# Autodesk Inventor assembly: Сборка
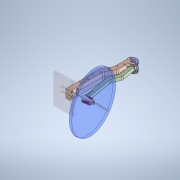
[picture p0: Inventor's stored thumbnail of the model, 180x180]
Saved by Autodesk Inventor 2021.2 (Build 252289000, 289)
## iProperties
Created: 2024-10-29
Part Number: Сборка
Document SubType Name: Assembly
Designer: barko
Author: barko
## Documents named in this file (14)
- C:\Users\barko\Desktop\Daniil\MIET\PID_controller\Mechanics\3D_model\Сборка.iam
- C:\Users\barko\Desktop\Daniil\MIET\PID_controller\Mechanics\3D_model\Ножка 1.ipt
- C:\Users\barko\Desktop\Daniil\MIET\PID_controller\Mechanics\3D_model\Ножка 2.ipt
- C:\Users\barko\Desktop\Daniil\MIET\PID_controller\Mechanics\3D_model\Скобка 1.ipt
- C:\Users\barko\Desktop\Daniil\MIET\PID_controller\Mechanics\3D_model\Скобка 2.ipt
- C:\Users\barko\Desktop\Daniil\MIET\PID_controller\Mechanics\3D_model\Фланец.ipt
- C:\Users\barko\Desktop\Daniil\MIET\PID_controller\Mechanics\3D_model\Луч.ipt
- C:\Users\barko\Desktop\Daniil\MIET\PID_controller\Mechanics\3D_model\Ложечка.ipt
- C:\Users\barko\Desktop\Daniil\MIET\PID_controller\Mechanics\3D_model\Моторчик.ipt
- C:\Users\barko\Desktop\Daniil\MIET\PID_controller\Mechanics\3D_model\Пропеллер.ipt
- C:\Users\barko\Documents\Inventor\Content Center Files\R2021\ru-RU\GOST 11738-84\Винт M3-6gx30 ГОСТ 11738-84.ipt
- C:\Users\barko\Documents\Inventor\Content Center Files\R2021\ru-RU\GOST 5916-70\Гайка M3-6H ГОСТ 5916-70.ipt
- C:\Users\barko\Documents\Inventor\Content Center Files\R2021\ru-RU\Nut GOST 15524-70\Гайка M4-6H ГОСТ 15524-70.ipt
- C:\Users\barko\Documents\Inventor\Content Center Files\R2021\ru-RU\GOST 11738-84\Винт M4-6gx25 ГОСТ 11738-84.ipt
## Components (25 placed, 13 different names)
1. Ножка 1:1 — Совмещение:1, Угол:1, Совмещение:2, Совмещение:3, Совмещение:4, Совмещение:5, Совмещение:6, Совмещение:7, Совмещение:8, Совмещение:9, Совмещение:10, Совмещение:11, Совмещение:12, Совмещение:13, Совмещение:14, Совмещение:15, Совмещение:16, Совмещение:18, Совмещение:20, Совмещение:22, Совмещение:24, Совмещение:26, Совмещение:28, Совмещение:33, Касательность:1, Касательность:2
2. Ножка 2:1 — Совмещение:17, Совмещение:19, Совмещение:21, Совмещение:23, Совмещение:25, Совмещение:27, Совмещение:29
3. Скобка 1:1 — Совмещение:34
4. Скобка 2:1
5. Фланец:1
6. Луч:1 — Вставка:3, Заподлицо:1, Совмещение:1, Угол:1
7. Ложечка:1 — Вставка:1
8. Моторчик:1 — Вставка:1, Вставка:2, Вставка:3
9. Пропеллер:1 — Вставка:2
10. Винт ГОСТ 11738-84 M 3x30:1 — Совмещение:2, Совмещение:3
11. Гайка ГОСТ 5916-70 M3:1 — Совмещение:16, Совмещение:17
12. Винт ГОСТ 11738-84 M 3x30:2 — Совмещение:4, Совмещение:5
13. Винт ГОСТ 11738-84 M 3x30:3 — Совмещение:6, Совмещение:7
14. Винт ГОСТ 11738-84 M 3x30:4 — Совмещение:8, Совмещение:9
15. Винт ГОСТ 11738-84 M 3x30:5 — Совмещение:10, Совмещение:11
16. Винт ГОСТ 11738-84 M 3x30:6 — Совмещение:12, Совмещение:13
17. Винт ГОСТ 11738-84 M 3x30:7 — Совмещение:14, Совмещение:15
18. Гайка ГОСТ 5916-70 M3:2 — Совмещение:18, Совмещение:19
19. Гайка ГОСТ 5916-70 M3:3 — Совмещение:20, Совмещение:21
20. Гайка ГОСТ 5916-70 M3:4 — Совмещение:22, Совмещение:23
21. Гайка ГОСТ 5916-70 M3:5 — Совмещение:24, Совмещение:25
22. Гайка ГОСТ 5916-70 M3:6 — Совмещение:26, Совмещение:27
23. Гайка ГОСТ 5916-70 M3:7 — Совмещение:28, Совмещение:29
24. Винт ГОСТ 11738-84 M 4x25:1 — Совмещение:33, Касательность:1, Касательность:2, Совмещение:35
25. Гайка ГОСТ 15524-70 M4:1 — Совмещение:34, Совмещение:35
## Relationships (39: Mate 32, Insert 3, Tangent 2, Flush 1, Angle 1)
- Вставка:1 [Insert]: Ложечка:1 ↔ Моторчик:1
- Вставка:2 [Insert] (2 mm): Моторчик:1 ↔ Пропеллер:1
- Вставка:3 [Insert]: Луч:1 ↔ Моторчик:1
- Заподлицо:1 [Flush]: Луч:1
- Совмещение:1 [Mate]: Ножка 1:1 ↔ Луч:1
- Угол:1 [Angle] (0 deg): Ножка 1:1 ↔ Луч:1
- Совмещение:2 [Mate]: Ножка 1:1 ↔ Винт ГОСТ 11738-84 M 3x30:1
- Совмещение:3 [Mate]: Ножка 1:1 ↔ Винт ГОСТ 11738-84 M 3x30:1
- Совмещение:4 [Mate]: Ножка 1:1 ↔ Винт ГОСТ 11738-84 M 3x30:2
- Совмещение:5 [Mate]: Ножка 1:1 ↔ Винт ГОСТ 11738-84 M 3x30:2
- Совмещение:6 [Mate]: Ножка 1:1 ↔ Винт ГОСТ 11738-84 M 3x30:3
- Совмещение:7 [Mate]: Ножка 1:1 ↔ Винт ГОСТ 11738-84 M 3x30:3
- Совмещение:8 [Mate]: Ножка 1:1 ↔ Винт ГОСТ 11738-84 M 3x30:4
- Совмещение:9 [Mate]: Ножка 1:1 ↔ Винт ГОСТ 11738-84 M 3x30:4
- Совмещение:10 [Mate]: Ножка 1:1 ↔ Винт ГОСТ 11738-84 M 3x30:5
- Совмещение:11 [Mate]: Ножка 1:1 ↔ Винт ГОСТ 11738-84 M 3x30:5
- Совмещение:12 [Mate]: Ножка 1:1 ↔ Винт ГОСТ 11738-84 M 3x30:6
- Совмещение:13 [Mate]: Ножка 1:1 ↔ Винт ГОСТ 11738-84 M 3x30:6
- Совмещение:14 [Mate]: Ножка 1:1 ↔ Винт ГОСТ 11738-84 M 3x30:7
- Совмещение:15 [Mate]: Ножка 1:1 ↔ Винт ГОСТ 11738-84 M 3x30:7
- Совмещение:16 [Mate]: Ножка 1:1 ↔ Гайка ГОСТ 5916-70 M3:1
- Совмещение:17 [Mate]: Ножка 2:1 ↔ Гайка ГОСТ 5916-70 M3:1
- Совмещение:18 [Mate]: Ножка 1:1 ↔ Гайка ГОСТ 5916-70 M3:2
- Совмещение:19 [Mate]: Ножка 2:1 ↔ Гайка ГОСТ 5916-70 M3:2
- Совмещение:20 [Mate]: Ножка 1:1 ↔ Гайка ГОСТ 5916-70 M3:3
- Совмещение:21 [Mate]: Ножка 2:1 ↔ Гайка ГОСТ 5916-70 M3:3
- Совмещение:22 [Mate]: Ножка 1:1 ↔ Гайка ГОСТ 5916-70 M3:4
- Совмещение:23 [Mate]: Ножка 2:1 ↔ Гайка ГОСТ 5916-70 M3:4
- Совмещение:24 [Mate]: Ножка 1:1 ↔ Гайка ГОСТ 5916-70 M3:5
- Совмещение:25 [Mate]: Ножка 2:1 ↔ Гайка ГОСТ 5916-70 M3:5
- Совмещение:26 [Mate]: Ножка 1:1 ↔ Гайка ГОСТ 5916-70 M3:6
- Совмещение:27 [Mate]: Ножка 2:1 ↔ Гайка ГОСТ 5916-70 M3:6
- Совмещение:28 [Mate]: Ножка 1:1 ↔ Гайка ГОСТ 5916-70 M3:7
- Совмещение:29 [Mate]: Ножка 2:1 ↔ Гайка ГОСТ 5916-70 M3:7
- Совмещение:33 [Mate]: Ножка 1:1 ↔ Винт ГОСТ 11738-84 M 4x25:1
- Касательность:1 [Tangent]: Ножка 1:1 ↔ Винт ГОСТ 11738-84 M 4x25:1
- Касательность:2 [Tangent]: Ножка 1:1 ↔ Винт ГОСТ 11738-84 M 4x25:1
- Совмещение:34 [Mate]: Скобка 1:1 ↔ Гайка ГОСТ 15524-70 M4:1
- Совмещение:35 [Mate]: Винт ГОСТ 11738-84 M 4x25:1 ↔ Гайка ГОСТ 15524-70 M4:1
